# Autodesk Inventor assembly: Inlet Assembly
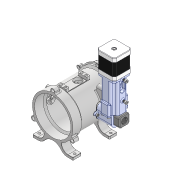
[picture p0: Inventor's stored thumbnail of the model, 180x180]
Saved by Autodesk Inventor 2020 (Build 240168000, 168)
## iProperties
Created: 2020-04-11
Part Number: Inlet Assembly
Document SubType Name: Assembly
Designer: John K
Author: John K
## Documents named in this file (4)
- C:\GrabCAD\MTL Ventilator Design\Breeze V2\Impeller Assembly\Inlet Assembly.iam
- C:\GrabCAD\MTL Ventilator Design\Breeze V2\Impeller Assembly\BRZ-P204.ipt
- C:\GrabCAD\MTL Ventilator Design\MTLV\Subassemblies\MTLV-S03.iam
- C:\GrabCAD\MTL Ventilator Design\Breeze V2\Inlet subassembly stuff - Angus\Butterfly valve.ipt
## Components (3 placed, 3 different names)
1. BRZ-P204:1 — Mate:1, Mate:2, Mate:3, Mate:4, Angle:1
2. MTLV-S03:1 [sub-assembly] — Mate:1, Mate:2, Mate:3
3. Butterfly valve:1 — Mate:4, Angle:1
## Relationships (5: Mate 4, Angle 1)
- Mate:1: BRZ-P204:1 ↔ MTLV-S03:1
- Mate:2: BRZ-P204:1 ↔ MTLV-S03:1
- Mate:3: BRZ-P204:1 ↔ MTLV-S03:1
- Mate:4: BRZ-P204:1 ↔ Butterfly valve:1
- Angle:1 (0 deg): BRZ-P204:1 ↔ Butterfly valve:1
